# Autodesk Inventor assembly: xtion_custom_assembly_v2_heatsink_mod
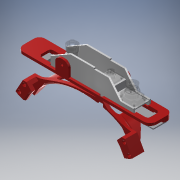
[picture p0: Inventor's stored thumbnail of the model, 180x180]
Saved by Autodesk Inventor 2017 (Build 210142000, 142)
## iProperties
Created: 2016-11-28
Part Number: xtion_custom_assembly_v2_heatsink_mod
Document SubType Name: Assembly
Designer: Ali
Author: Ali
## Documents named in this file (8)
- C:\Users\Alistair\Dropbox\Work\HeadSLAM\prototype-2\xtion_custom_assembly_v2_heatsink_mod.iam
- C:\Users\Alistair\Dropbox\Work\HeadSLAM\prototype-2\head_mount_v2.ipt
- C:\Users\Alistair\Dropbox\Work\HeadSLAM\xtion-internal\xtion_mainboard.ipt
- C:\Users\Alistair\Dropbox\Work\HeadSLAM\xtion-internal\xtion_ir_cam.ipt
- C:\Users\Alistair\Dropbox\Work\HeadSLAM\xtion-internal\xtion_projector.ipt
- C:\Users\Alistair\Dropbox\Work\HeadSLAM\xtion-internal\xtion_rgb_cam.ipt
- C:\Users\Alistair\Dropbox\Work\HeadSLAM\prototype-2\xtion_heatsink_mod.ipt
- C:\Users\Alistair\Dropbox\Work\HeadSLAM\xtion_custom_heatsink_mount.ipt
## Components (7 placed, 7 different names)
1. head_mount_v2:1 — Rigid:1, Flush:1
2. xtion_mainboard:1 — Rigid:1
3. xtion_ir_cam:1 — Rigid:4
4. xtion_projector:1 — Rigid:2
5. xtion_rgb_cam:1 — Rigid:3
6. xtion_heatsink_mod:1 — Rigid:2, Rigid:3, Rigid:4
7. xtion_custom_heatsink_mount:1 — Flush:1
## Relationships (5: WeldJoint 4, Flush 1)
- Rigid:1 [WeldJoint]: head_mount_v2:1 ↔ xtion_mainboard:1
- Rigid:2 [WeldJoint]: xtion_projector:1 ↔ xtion_heatsink_mod:1
- Rigid:3 [WeldJoint]: xtion_rgb_cam:1 ↔ xtion_heatsink_mod:1
- Rigid:4 [WeldJoint]: xtion_ir_cam:1 ↔ xtion_heatsink_mod:1
- Flush:1: head_mount_v2:1 ↔ xtion_custom_heatsink_mount:1
